# Autodesk Inventor assembly: outer
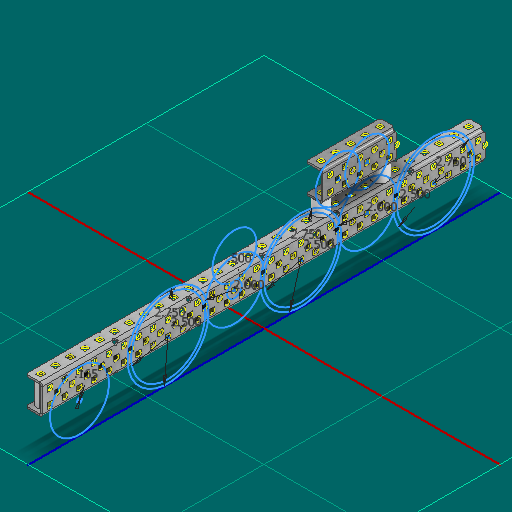
[picture p0: Inventor's stored thumbnail of the model, 512x512]
Saved by Autodesk Inventor 2025 (Build 290162000, 162)
## iProperties
Created: 2024-10-02
Part Number: outer
Document SubType Name: Assembly
Designer: Averey Ku
Author: Averey Ku
## Documents named in this file (8)
- C:\Users\avere\vex_robotics_high_stakes\hardware\cad\bots\high_stakes_v2\chassis\drivebay\outer.iam
- C:\Users\avere\vex_robotics_high_stakes\hardware\cad\robpros_cad_lib\Structure\C Channel\Aluminum 1x2x1\Alu C 1x2x1x30.ipt
- C:\Users\avere\vex_robotics_high_stakes\hardware\cad\robpros_cad_lib\Motion\Shaft LS\Bearing Flat Low Profile.ipt
- C:\Users\avere\vex_robotics_high_stakes\hardware\cad\robpros_cad_lib\Motion\Spacers\Spacer Nylon .500 OD\NSpacer White .500 OD x .500.ipt
- D:\vex_robotics_high_stakes\hardware\cad\robpros_cad_lib\Motion\Spacers\Spacer Nylon .500 OD.ipt
- C:\Users\avere\vex_robotics_high_stakes\hardware\cad\robpros_cad_lib\Structure\C Channel\Aluminum 1x2x1\Alu C 1x2x1x5.ipt
- C:\Users\avere\vex_robotics_high_stakes\hardware\cad\VEX-CAD-Inventor\Structure\Standoff\Standoff .875.ipt
- D:\vex_robotics_high_stakes\hardware\cad\VEX-CAD-Inventor\Structure\Standoff.ipt
## Components (12 placed, 5 different names)
1. Alu C 1x2x1x30:2 — Insert:1, Mate:1, Insert:2, Mate:2, Insert:3, Mate:3, Insert:4, Mate:4, Insert:5, Mate:5, Insert:6, Insert:7, Insert:20, Insert:21
2. Bearing Flat Low Profile:1 — Insert:2, Mate:2
3. Bearing Flat Low Profile:2 — Insert:3, Mate:3
4. Bearing Flat Low Profile:3 — Insert:1, Mate:1
5. Bearing Flat Low Profile:4 — Insert:5, Mate:5
6. Bearing Flat Low Profile:5 — Insert:4, Mate:4
7. NSpacer White .500 OD x .500:1 — Insert:7, Insert:18
8. NSpacer White .500 OD x .500:2 — Insert:6, Mate:11
9. Bearing Flat Low Profile:6 — Insert:19, Mate:12
10. Alu C 1x2x1x5:1 — Insert:18, Mate:11, Insert:19, Mate:12
11. Standoff .875:1 — Insert:20
12. Standoff .875:2 — Insert:21
## Relationships (18: Insert 11, Mate 7)
- Insert:1: Alu C 1x2x1x30:2 ↔ Bearing Flat Low Profile:3
- Mate:1: Alu C 1x2x1x30:2 ↔ Bearing Flat Low Profile:3
- Insert:2: Alu C 1x2x1x30:2 ↔ Bearing Flat Low Profile:1
- Mate:2: Alu C 1x2x1x30:2 ↔ Bearing Flat Low Profile:1
- Insert:3: Alu C 1x2x1x30:2 ↔ Bearing Flat Low Profile:2
- Mate:3: Alu C 1x2x1x30:2 ↔ Bearing Flat Low Profile:2
- Insert:4: Alu C 1x2x1x30:2 ↔ Bearing Flat Low Profile:5
- Mate:4: Alu C 1x2x1x30:2 ↔ Bearing Flat Low Profile:5
- Insert:5: Alu C 1x2x1x30:2 ↔ Bearing Flat Low Profile:4
- Mate:5: Alu C 1x2x1x30:2 ↔ Bearing Flat Low Profile:4
- Insert:6: Alu C 1x2x1x30:2 ↔ NSpacer White .500 OD x .500:2
- Insert:7: Alu C 1x2x1x30:2 ↔ NSpacer White .500 OD x .500:1
- Insert:18: NSpacer White .500 OD x .500:1 ↔ Alu C 1x2x1x5:1
- Mate:11: NSpacer White .500 OD x .500:2 ↔ Alu C 1x2x1x5:1
- Insert:19: Bearing Flat Low Profile:6 ↔ Alu C 1x2x1x5:1
- Mate:12: Bearing Flat Low Profile:6 ↔ Alu C 1x2x1x5:1
- Insert:20: Alu C 1x2x1x30:2 ↔ Standoff .875:1
- Insert:21: Alu C 1x2x1x30:2 ↔ Standoff .875:2
